# Autodesk Inventor assembly: leg_left
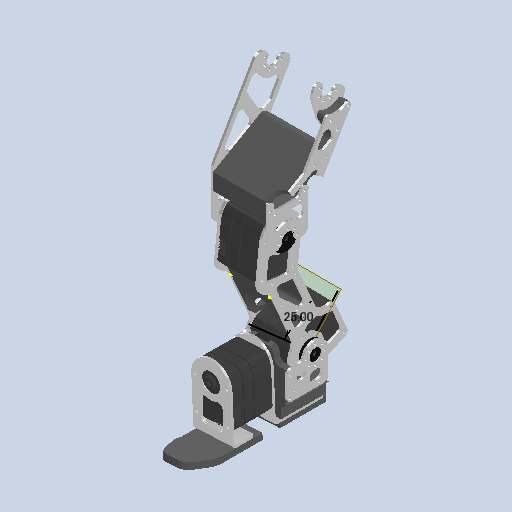
[picture p0: Inventor's stored thumbnail of the model, 512x512]
Saved by Autodesk Inventor 2026.1 (Build 301233020, 233B)
## iProperties
Created: 2024-10-11
Part Number: leg_left
Document SubType Name: Assembly
Designer: hibik
Author: hibik
## Documents named in this file (4)
- C:\Users\hibik\Documents\Robomech\HR\Eglantyne_mark2\hard\leg\leg_left.iam
- C:\Users\hibik\Documents\Robomech\HR\Eglantyne_mark2\hard\leg\leg_upper_left.iam
- C:\Users\hibik\Documents\Robomech\HR\Eglantyne_mark2\hard\leg\leg_under.iam
- C:\Users\hibik\Documents\Robomech\HR\Eglantyne_mark2\hard\leg\toe.iam
## Components (3 placed, 3 different names)
1. leg_upper_left:1 [sub-assembly] — フラッシュ:1, メイト:1, フラッシュ:2, 挿入:1
2. leg_under:1 [sub-assembly] — 挿入:1, 挿入:2
3. toe:1 [sub-assembly] — 挿入:2
## Relationships (5: Flush 2, Insert 2, Mate 1)
- フラッシュ:1 [Flush]: leg_upper_left:1
- メイト:1 [Mate]: leg_upper_left:1
- フラッシュ:2 [Flush]: leg_upper_left:1
- 挿入:1 [Insert]: leg_upper_left:1 ↔ leg_under:1
- 挿入:2 [Insert]: leg_under:1 ↔ toe:1
